# Autodesk Inventor assembly: FarmBot
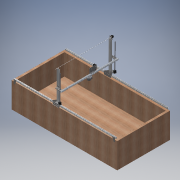
[picture p0: Inventor's stored thumbnail of the model, 180x180]
Saved by Autodesk Inventor 2017 (Build 210142000, 142)
## iProperties
Created: 2016-12-12
Part Number: FarmBot
Document SubType Name: Assembly
Designer: umr
Author: umr
## Documents named in this file (6)
- D:\SeniorProject\Models2\FarmBot.iam
- D:\SeniorProject\Models2\BedAssembly\BedAseembly.iam
- D:\SeniorProject\Models2\Head\HeadSlider.iam
- D:\SeniorProject\Models2\Gantry\GantryDown.iam
- D:\SeniorProject\Models2\Gantry\GantryUp.iam
- D:\SeniorProject\Models2\Case\Case.iam
## Components (5 placed, 5 different names)
1. BedAseembly:2 [sub-assembly] — Mate:8, Flush:2, Flush:3, Mate:9, Tangent:1, Tangent:2
2. HeadSlider:1 [sub-assembly] — Mate:6, Mate:7
3. GantryDown:1 [sub-assembly] — Mate:3, Mate:5, Mate:9, Tangent:1, Tangent:2
4. GantryUp:1 [sub-assembly] — Mate:3, Mate:5, Mate:6, Mate:7
5. Case:1 [sub-assembly] — Mate:8, Flush:2, Flush:3
## Relationships (10: Mate 6, Flush 2, Tangent 2)
- Mate:3: GantryDown:1 ↔ GantryUp:1
- Mate:5: GantryDown:1 ↔ GantryUp:1
- Mate:6: HeadSlider:1 ↔ GantryUp:1
- Mate:7: HeadSlider:1 ↔ GantryUp:1
- Mate:8: BedAseembly:2 ↔ Case:1
- Flush:2 (-150 mm): BedAseembly:2 ↔ Case:1
- Flush:3 (-100 mm): BedAseembly:2 ↔ Case:1
- Mate:9: BedAseembly:2 ↔ GantryDown:1
- Tangent:1: BedAseembly:2 ↔ GantryDown:1
- Tangent:2: BedAseembly:2 ↔ GantryDown:1
